# Autodesk Inventor assembly: ensamble_general
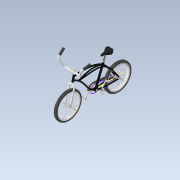
[picture p0: Inventor's stored thumbnail of the model, 180x180]
Saved by Autodesk Inventor 2021 (Build 250183000, 183)
## iProperties
Created: 2021-04-10
Part Number: ensamble_general
Document SubType Name: Assembly
Designer: j2seb
Author: j2seb
## Documents named in this file (9)
- C:\Git\Proyecto_APM\02 Inventor\ensamble_general.iam
- C:\Git\Proyecto_APM\02 Inventor\Marco_Bicicleta.iam
- C:\Git\Proyecto_APM\02 Inventor\Manubrio\Manubrio.ipt
- C:\Git\Proyecto_APM\02 Inventor\sillin.iam
- C:\Git\Proyecto_APM\02 Inventor\caja_pedalera.iam
- C:\Git\Proyecto_APM\02 Inventor\Transmision\Cadena.iam
- C:\Git\Proyecto_APM\02 Inventor\cubrecadena.ipt
- C:\Git\Proyecto_APM\02 Inventor\llanta trasera.iam
- C:\Git\Proyecto_APM\02 Inventor\llanta delantera.iam
## Components (8 placed, 8 different names)
1. Marco_Bicicleta:1 [sub-assembly] — Coincidencia:3, Flush:1, Cylindrical:2, Mate:5, Coincidencia:6, Coincidencia:7, Mate:8, Mate:9, Coincidencia:16, Coincidencia:19
2. Manubrio:1 — Flush:1, Coincidencia:19
3. sillin:1 [sub-assembly] — Cylindrical:2, Mate:5
4. caja_pedalera:1 [sub-assembly] — Coincidencia:6, Coincidencia:7
5. Cadena:1 [sub-assembly] — Mate:12
6. cubrecadena:1 — Mate:15
7. llanta trasera:1 [sub-assembly] — Coincidencia:16
8. llanta delantera:1 [sub-assembly] — Coincidencia:18
## Relationships (15: Mate 12, Angle 1, Flush 1, CylindricalJoint 1)
- [Mate]: Marco_Bicicleta:1 ↔ llanta trasera:1
- Coincidencia:3 [Mate]: Marco_Bicicleta:1
- Ángulo:1 [Angle] (0 deg)
- Flush:1 (-55.052 mm): Marco_Bicicleta:1 ↔ Manubrio:1
- Cylindrical:2: Marco_Bicicleta:1 ↔ sillin:1
- Mate:5 (-50 mm): Marco_Bicicleta:1 ↔ sillin:1
- Coincidencia:6 [Mate]: Marco_Bicicleta:1 ↔ caja_pedalera:1
- Coincidencia:7 [Mate]: Marco_Bicicleta:1 ↔ caja_pedalera:1
- Mate:8: Marco_Bicicleta:1
- Mate:9: Marco_Bicicleta:1
- Mate:12: Cadena:1
- Mate:15: cubrecadena:1
- Coincidencia:16 [Mate]: Marco_Bicicleta:1 ↔ llanta trasera:1
- Coincidencia:18 [Mate]: llanta delantera:1
- Coincidencia:19 [Mate]: Marco_Bicicleta:1 ↔ Manubrio:1
## Named parameters: DExtTub = 42.164 mm, DintTub = 35.052 mm, DIntTubTen = 28 mm, DAguUniMarcoLlanta = 4 mm
